# Autodesk Inventor assembly: Pok Mk1
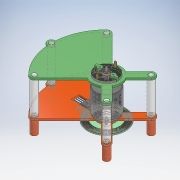
[picture p0: Inventor's stored thumbnail of the model, 180x180]
Saved by Autodesk Inventor 2018.2 (Build 222227000, 227)
## iProperties
Created: 2018-02-07
Part Number: Pok Mk1
Document SubType Name: Assembly
Designer: Moochster
Author: Moochster
## Documents named in this file (10)
- C:\Users\Moochster\OneDrive\Documents\2018 UBC\ELEC 391\Controller\CAD\Pok Mk1.iam
- C:\Users\Moochster\OneDrive\Documents\2018 UBC\ELEC 391\Controller\CAD\JD5B-2655W-R.ipt
- C:\Users\Moochster\OneDrive\Documents\2018 UBC\ELEC 391\Controller\CAD\Encoder Wheel (G16).ipt
- C:\Users\Moochster\OneDrive\Documents\2018 UBC\ELEC 391\Controller\CAD\Pok Yaw Motor Face Mount.ipt
- C:\Users\Moochster\OneDrive\Documents\2018 UBC\ELEC 391\Controller\CAD\Pok Washer I2mmO5mm.ipt
- C:\Users\Moochster\OneDrive\Documents\2018 UBC\ELEC 391\Controller\CAD\Shaft Washer.ipt
- C:\Users\Moochster\OneDrive\Documents\2018 UBC\ELEC 391\Controller\CAD\GP1A52HRJ00F (Large slot detector).ipt
- C:\Users\Moochster\OneDrive\Documents\2018 UBC\ELEC 391\Controller\CAD\Pok X-Carriage Bottom Support.ipt
- C:\Users\Moochster\OneDrive\Documents\2018 UBC\ELEC 391\Controller\CAD\Pok X-Carriage Top Support.ipt
- C:\Users\Moochster\OneDrive\Documents\2018 UBC\ELEC 391\Controller\CAD\Pok Y-Carriage.ipt
## Components (19 placed, 9 different names)
1. JD5B-2655W-R:1 — Mate:1, Mate:2, Mate:7, Mate:8, Mate:11, Mate:29, Mate:30, Mate:32
2. Encoder Wheel (G16):1 — Mate:2, Mate:13, Mate:27, Angle:3
3. Pok Yaw Motor Face Mount:1 — Angle:1, Mate:29, Mate:30, Mate:31, Insert:4, Insert:6, Insert:7, Insert:8, Insert:11
4. Pok Washer I2mmO5mm:1 — Mate:7, Mate:31
5. Pok Washer I2mmO5mm:2 — Mate:8
6. Shaft Washer:1 — Mate:11, Mate:27, Angle:3
7. GP1A52HRJ00F (Large slot detector):1 — Mate:12, Flush:1, Flush:2, Mate:13
8. GP1A52HRJ00F (Large slot detector):2 — Mate:12, Flush:1, Flush:2, Angle:2
9. Pok X-Carriage Bottom Support:1 — Insert:2, Insert:4
10. Pok X-Carriage Bottom Support:2 — Mate:28, Insert:3, Insert:6
11. Pok X-Carriage Bottom Support:3 — Insert:8, Insert:10
12. Pok X-Carriage Bottom Support:4 — Insert:7, Insert:9
13. Pok X-Carriage Bottom Support:5 — Insert:1, Insert:11
14. Pok X-Carriage Top Support:1 — Insert:2
15. Pok X-Carriage Top Support:2 — Insert:1, Mate:33
16. Pok X-Carriage Top Support:3 — Insert:3
17. Pok X-Carriage Top Support:4 — Insert:10
18. Pok X-Carriage Top Support:5 — Insert:9
19. Pok Y-Carriage:1 — Mate:32, Mate:33
## Relationships (29: Mate 14, Insert 10, Angle 3, Flush 2)
- Mate:1: JD5B-2655W-R:1
- Mate:2: JD5B-2655W-R:1 ↔ Encoder Wheel (G16):1
- Mate:7: JD5B-2655W-R:1 ↔ Pok Washer I2mmO5mm:1
- Mate:8: JD5B-2655W-R:1 ↔ Pok Washer I2mmO5mm:2
- Mate:11: JD5B-2655W-R:1 ↔ Shaft Washer:1
- Mate:12: GP1A52HRJ00F (Large slot detector):1 ↔ GP1A52HRJ00F (Large slot detector):2
- Flush:1: GP1A52HRJ00F (Large slot detector):1 ↔ GP1A52HRJ00F (Large slot detector):2
- Flush:2: GP1A52HRJ00F (Large slot detector):1 ↔ GP1A52HRJ00F (Large slot detector):2
- Mate:13 (0.7 mm): Encoder Wheel (G16):1 ↔ GP1A52HRJ00F (Large slot detector):1
- Angle:1 (0 deg): Pok Yaw Motor Face Mount:1
- Angle:2 (0 deg): GP1A52HRJ00F (Large slot detector):2
- Mate:27: Encoder Wheel (G16):1 ↔ Shaft Washer:1
- Mate:28: Pok X-Carriage Bottom Support:2
- Angle:3 (0 deg): Encoder Wheel (G16):1 ↔ Shaft Washer:1
- Insert:1 (0.1 mm): Pok X-Carriage Bottom Support:5 ↔ Pok X-Carriage Top Support:2
- Insert:2 (0.1 mm): Pok X-Carriage Bottom Support:1 ↔ Pok X-Carriage Top Support:1
- Insert:3 (0.1 mm): Pok X-Carriage Bottom Support:2 ↔ Pok X-Carriage Top Support:3
- Mate:29: JD5B-2655W-R:1 ↔ Pok Yaw Motor Face Mount:1
- Mate:30: JD5B-2655W-R:1 ↔ Pok Yaw Motor Face Mount:1
- Mate:31 (0.1 mm): Pok Yaw Motor Face Mount:1 ↔ Pok Washer I2mmO5mm:1
- Insert:4 (0.1 mm): Pok Yaw Motor Face Mount:1 ↔ Pok X-Carriage Bottom Support:1
- Insert:6 (0.1 mm): Pok Yaw Motor Face Mount:1 ↔ Pok X-Carriage Bottom Support:2
- Insert:7 (0.1 mm): Pok Yaw Motor Face Mount:1 ↔ Pok X-Carriage Bottom Support:4
- Insert:8 (0.1 mm): Pok Yaw Motor Face Mount:1 ↔ Pok X-Carriage Bottom Support:3
- Insert:9 (0.1 mm): Pok X-Carriage Bottom Support:4 ↔ Pok X-Carriage Top Support:5
- Insert:10 (0.1 mm): Pok X-Carriage Bottom Support:3 ↔ Pok X-Carriage Top Support:4
- Mate:32: JD5B-2655W-R:1 ↔ Pok Y-Carriage:1
- Insert:11 (0.1 mm): Pok Yaw Motor Face Mount:1 ↔ Pok X-Carriage Bottom Support:5
- Mate:33: Pok X-Carriage Top Support:2 ↔ Pok Y-Carriage:1
